# Autodesk Inventor assembly: Horquilla
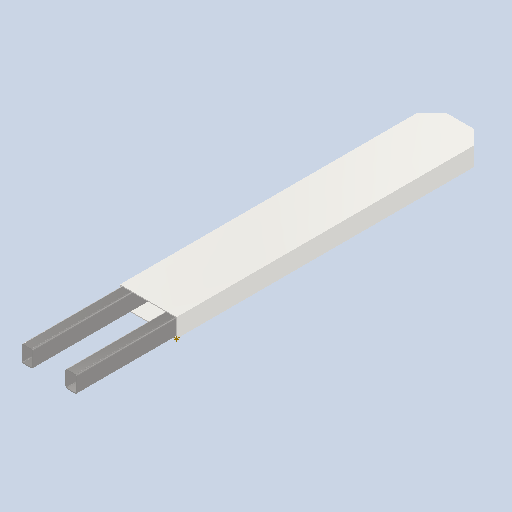
[picture p0: Inventor's stored thumbnail of the model, 512x512]
Saved by Autodesk Inventor 2022.1 (Build 261234000, 234)
## iProperties
Created: 2021-09-10
Part Number: Horquilla
Document SubType Name: Assembly
Designer: seb_0
Author: seb_0
## Documents named in this file (6)
- C:\Users\seb_0\Desktop\RobotPallet_v3\Horquillas\Horquilla.iam
- C:\Users\seb_0\Desktop\RobotPallet_v3\Horquillas\Horquilla_Base.ipt
- C:\Users\seb_0\Desktop\RobotPallet_v3\Horquillas\Horquilla_Cubierta.ipt
- C:\Users\seb_0\Desktop\RobotPallet_v3\Horquillas\Rueda_Soporte.ipt
- C:\Users\seb_0\Desktop\RobotPallet_v3\Horquillas\Rueda_Rueda.ipt
- C:\Users\seb_0\Desktop\RobotPallet_v3\Horquillas\DIN 59 410 - 60x40x2.9-1400.ipt
## Components (6 placed, 5 different names)
1. Horquilla_Base:1 — Coincidencia:1, Coincidencia:2, Coincidencia:3, Nivelación:1, Nivelación:2, Coincidencia:4, Coincidencia:15, Coincidencia:17, Coincidencia:18, Nivelación:5, Nivelación:6, Nivelación:7, Nivelación:8, Coincidencia:19
2. Horquilla_Cubierta:1 — Nivelación:1, Nivelación:2, Coincidencia:19
3. Rueda_Soporte:1 — Coincidencia:4, Coincidencia:5, Coincidencia:15
4. Rueda_Rueda:1 — Coincidencia:5
5. DIN 59 410 - 60x40x2.9-1400:1 — Coincidencia:18, Nivelación:5, Nivelación:8
6. DIN 59 410 - 60x40x2.9-1400:2 — Coincidencia:17, Nivelación:6, Nivelación:7
## Relationships (15: Mate 9, Flush 6)
- Coincidencia:1 [Mate]: Horquilla_Base:1
- Coincidencia:2 [Mate]: Horquilla_Base:1
- Coincidencia:3 [Mate]: Horquilla_Base:1
- Nivelación:1 [Flush]: Horquilla_Base:1 ↔ Horquilla_Cubierta:1
- Nivelación:2 [Flush]: Horquilla_Base:1 ↔ Horquilla_Cubierta:1
- Coincidencia:4 [Mate]: Horquilla_Base:1 ↔ Rueda_Soporte:1
- Coincidencia:5 [Mate]: Rueda_Soporte:1 ↔ Rueda_Rueda:1
- Coincidencia:15 [Mate]: Horquilla_Base:1 ↔ Rueda_Soporte:1
- Coincidencia:17 [Mate]: Horquilla_Base:1 ↔ DIN 59 410 - 60x40x2.9-1400:2
- Coincidencia:18 [Mate]: Horquilla_Base:1 ↔ DIN 59 410 - 60x40x2.9-1400:1
- Nivelación:5 [Flush] (2.5 mm): Horquilla_Base:1 ↔ DIN 59 410 - 60x40x2.9-1400:1
- Nivelación:6 [Flush] (2.5 mm): Horquilla_Base:1 ↔ DIN 59 410 - 60x40x2.9-1400:2
- Nivelación:7 [Flush] (50 mm): Horquilla_Base:1 ↔ DIN 59 410 - 60x40x2.9-1400:2
- Nivelación:8 [Flush] (50 mm): Horquilla_Base:1 ↔ DIN 59 410 - 60x40x2.9-1400:1
- Coincidencia:19 [Mate]: Horquilla_Base:1 ↔ Horquilla_Cubierta:1
